# Autodesk Inventor assembly: WallEAssembly
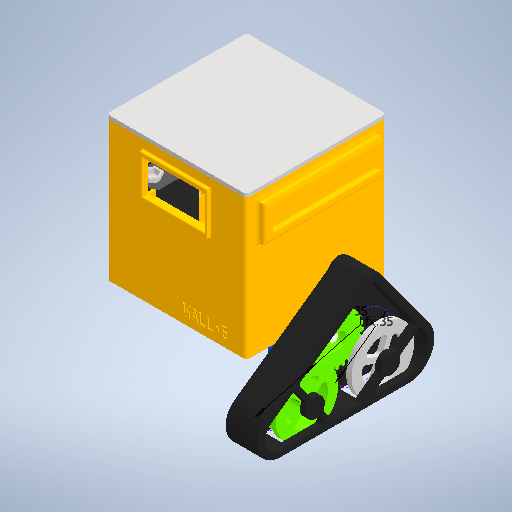
[picture p0: Inventor's stored thumbnail of the model, 512x512]
Saved by Autodesk Inventor 2025.2 (Build 292293000, 293)
## iProperties
Created: 2025-01-25
Part Number: WallEAssembly
Document SubType Name: Assembly
Designer: andre
Author: andre
## Documents named in this file (10)
- C:\Users\andre\Documents\GitHub\Handshake\Hardware\Proto2-WallE\WallEAssembly.iam
- C:\Users\andre\Documents\GitHub\Handshake\Hardware\Proto2-WallE\WallEBody.ipt
- C:\Users\andre\Documents\GitHub\Handshake\Hardware\Common\PCBModel.ipt
- C:\Users\andre\Documents\GitHub\Handshake\Hardware\Common\Battery_9V\Battery_9V\Battery_9V.ipt
- C:\Users\andre\Documents\GitHub\Handshake\Hardware\Proto2-WallE\TreadAssembly.iam
- C:\Users\andre\Documents\GitHub\Handshake\Hardware\Common\Servo Motor SG90.ipt
- C:\Users\andre\Documents\GitHub\Handshake\Hardware\Proto2-WallE\WallEAssembly\Design Accelerator\Spur Gears1.iam
- C:\Users\andre\Documents\GitHub\Handshake\Hardware\Proto2-WallE\ BodyLid.ipt
- C:\Users\andre\Documents\GitHub\Handshake\Hardware\Proto2-WallE\Wheel.ipt
- C:\Users\andre\Documents\GitHub\Handshake\Hardware\Proto2-WallE\BodyLid.ipt
## Components (8 placed, 8 different names)
1. WallEBody:1 — Mate:1, Angle:1, Mate:2, Mate:3, Mate:4, Angle:2, Mate:5, Mate:6, Mate:8, Mate:9, Flush:1, Flush:2
2. PCBModel:1 — Mate:1, Angle:1, Mate:2
3. Battery_9V:1 — Mate:3, Mate:8
4. TreadAssembly:1 [sub-assembly] — Mate:4, Angle:2, Mate:5, Mate:6, Mate:7, Mate:12
5. Servo Motor SG90:1 — Mate:7, Mate:9, Mate:10, Mate:11
6. Spur Gears:1 [sub-assembly] — Mate:10, Mate:11
7. BodyLid:1 — Flush:1, Flush:2
8. Wheel:1 — Mate:12
## Relationships (16: Mate 12, Angle 2, Flush 2)
- Mate:1 (2.3 mm): WallEBody:1 ↔ PCBModel:1
- Angle:1 (0 deg): WallEBody:1 ↔ PCBModel:1
- Mate:2: WallEBody:1 ↔ PCBModel:1
- Mate:3: WallEBody:1 ↔ Battery_9V:1
- Mate:4: WallEBody:1 ↔ TreadAssembly:1
- Angle:2 (0 deg): WallEBody:1 ↔ TreadAssembly:1
- Mate:5: WallEBody:1 ↔ TreadAssembly:1
- Mate:6: WallEBody:1 ↔ TreadAssembly:1
- Mate:7: TreadAssembly:1 ↔ Servo Motor SG90:1
- Mate:8: WallEBody:1 ↔ Battery_9V:1
- Mate:9: WallEBody:1 ↔ Servo Motor SG90:1
- Mate:10: Servo Motor SG90:1 ↔ Spur Gears:1
- Mate:11: Servo Motor SG90:1 ↔ Spur Gears:1
- Flush:1: WallEBody:1 ↔ BodyLid:1
- Flush:2: WallEBody:1 ↔ BodyLid:1
- Mate:12: TreadAssembly:1 ↔ Wheel:1
